# Autodesk Inventor assembly: Assembly_cellSTORM_inverted_opticmodule_v0
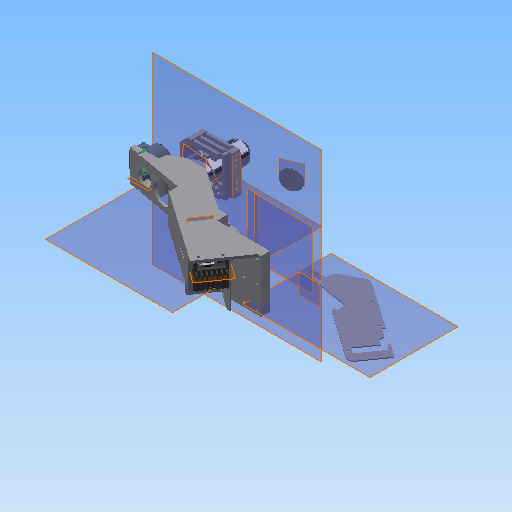
[picture p0: Inventor's stored thumbnail of the model, 512x512]
Saved by Autodesk Inventor 2019.4 (Build 234330000, 330)
## iProperties
Created: 2020-11-06
Part Number: Assembly_cellSTORM_inverted_opticmodule_v0
Document SubType Name: Assembly
Designer: diederichbenedict
Author: diederichbenedict
## Documents named in this file (13)
- C:\Users\diederichbenedict\Dropbox\Dokumente\Promotion\PROJECTS\STORMoChip\GITHUB\CAD\cellSTORM_inverted\Workspace\Assembly_cellSTORM_opticmodule_v0.iam
- C:\Users\diederichbenedict\Dropbox\Dokumente\Promotion\PROJECTS\STORMoChip\GITHUB\CAD\cellSTORM_inverted\Workspace\00_Microscope_Objective.ipt
- C:\Users\diederichbenedict\Dropbox\Dokumente\Promotion\PROJECTS\STORMoChip\GITHUB\CAD\cellSTORM_inverted\Workspace\PF10-03-P01-Step.ipt
- C:\Users\diederichbenedict\Dropbox\Dokumente\Promotion\PROJECTS\STORMoChip\GITHUB\CAD\cellSTORM_inverted\Workspace\00_Alvium_Step_USB90_S-Mount_ClosedHousing_2019-Mar-28.ipt
- C:\Users\diederichbenedict\Dropbox\Dokumente\Promotion\PROJECTS\STORMoChip\GITHUB\CAD\cellSTORM_inverted\Workspace\AC254-050-A-ML-Step.ipt
- C:\Users\diederichbenedict\Dropbox\Dokumente\Promotion\PROJECTS\STORMoChip\GITHUB\CAD\cellSTORM_inverted\Workspace\10_Filteslide_25mm.ipt
- C:\Users\diederichbenedict\Dropbox\Dokumente\Promotion\PROJECTS\STORMoChip\GITHUB\CAD\cellSTORM_inverted\Workspace\cellSTORM_inverted_opticsmodule_v0.ipt
- C:\Users\diederichbenedict\Dropbox\Dokumente\Promotion\PROJECTS\STORMoChip\GITHUB\CAD\cellSTORM_inverted\Workspace\00_Stepper_Motor_28BYJ-48.0013.ipt
- C:\Users\diederichbenedict\Dropbox\Dokumente\Promotion\PROJECTS\STORMoChip\GITHUB\CAD\cellSTORM_inverted\Workspace\10_Lensslide_f50mm.ipt
- C:\Users\diederichbenedict\Dropbox\Dokumente\Promotion\PROJECTS\STORMoChip\GITHUB\CAD\cellSTORM_inverted\Workspace\cellSTORM_inverted_opticsmodule_lid.ipt
- C:\Users\diederichbenedict\Dropbox\Dokumente\Promotion\PROJECTS\STORMoChip\GITHUB\CAD\cellSTORM_inverted\Workspace\cellSTORM_v5_focussingunit_1.ipt
- C:\Users\diederichbenedict\Dropbox\Dokumente\Promotion\PROJECTS\STORMoChip\GITHUB\CAD\cellSTORM_inverted\Workspace\cellSTORM_inverted_objectiveadapter.ipt
- C:\Users\diederichbenedict\Dropbox\Dokumente\Promotion\PROJECTS\STORMoChip\GITHUB\CAD\cellSTORM_inverted\Workspace\cellSTORM_lightpath_upright.ipt
## Components (12 placed, 12 different names)
1. 00_Alvium_Step_USB90_S-Mount_ClosedHousing_2019-Mar-28:1 — Angle:1, Mate:8, Mate:9, Angle:4
2. 00_Stepper_Motor_28BYJ-48.0013:1
3. 10_Filteslide_25mm:1 — Angle:1, Angle:3, Mate:8
4. cellSTORM_inverted_opticsmodule_v0:1 — Flush:1, Insert:7, Flush:7
5. 10_Lensslide_f50mm:1 — Insert:8, Flush:7
6. AC254-050-A-ML-Step:1 — Insert:7, Insert:8
7. cellSTORM_inverted_opticsmodule_lid:1
8. cellSTORM_lightpath_upright:1 — Mate:9, Insert:9, Insert:10, Angle:4
9. PF10-03-P01-Step:1 — Insert:9
10. 00_Microscope_Objective:1 — Insert:10, Mate:10
11. cellSTORM_inverted_objectiveadapter:1
12. cellSTORM_v5_focussingunit_1:1 — Mate:10
## Relationships (12: Insert 4, Angle 3, Mate 3, Flush 2)
- Angle:1 (0 deg): 00_Alvium_Step_USB90_S-Mount_ClosedHousing_2019-Mar-28:1 ↔ 10_Filteslide_25mm:1
- Flush:1: cellSTORM_inverted_opticsmodule_v0:1
- Angle:3 (0 deg): 10_Filteslide_25mm:1
- Mate:8 (8 mm): 00_Alvium_Step_USB90_S-Mount_ClosedHousing_2019-Mar-28:1 ↔ 10_Filteslide_25mm:1
- Insert:7 (-7 mm): cellSTORM_inverted_opticsmodule_v0:1 ↔ AC254-050-A-ML-Step:1
- Insert:8: 10_Lensslide_f50mm:1 ↔ AC254-050-A-ML-Step:1
- Flush:7: cellSTORM_inverted_opticsmodule_v0:1 ↔ 10_Lensslide_f50mm:1
- Mate:9: 00_Alvium_Step_USB90_S-Mount_ClosedHousing_2019-Mar-28:1 ↔ cellSTORM_lightpath_upright:1
- Insert:9: cellSTORM_lightpath_upright:1 ↔ PF10-03-P01-Step:1
- Insert:10: cellSTORM_lightpath_upright:1 ↔ 00_Microscope_Objective:1
- Angle:4 (180 deg): 00_Alvium_Step_USB90_S-Mount_ClosedHousing_2019-Mar-28:1 ↔ cellSTORM_lightpath_upright:1
- Mate:10: 00_Microscope_Objective:1 ↔ cellSTORM_v5_focussingunit_1:1
